# Autodesk Inventor assembly: Pakiet_zagrzany_same_ogniwa
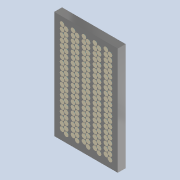
[picture p0: Inventor's stored thumbnail of the model, 180x180]
Saved by Autodesk Inventor 2021.3 (Build 253353000, 353)
## iProperties
Created: 2023-05-23
Part Number: Pakiet_zagrzany_same_ogniwa
Document SubType Name: Assembly
Designer: User
Author: User
## Documents named in this file (3)
- E:\Inventor\Projekty\Modele Robotyzacja Procesów\Pakiet_zagrzany_same_ogniwa.iam
- E:\Inventor\Projekty\Modele Robotyzacja Procesów\Model_Sita.ipt
- E:\Inventor\Projekty\Modele Robotyzacja Procesów\Model_Ogniwa.ipt
## Components (201 placed, 2 different names)
1. Model_Sita:1 — Zestawiające:1, Równoległe:1, Zestawiające:2, Równoległe:2
2. Model_Ogniwa:1 — Zestawiające:1, Równoległe:1
3. Model_Ogniwa:2
4. Model_Ogniwa:3
5. Model_Ogniwa:4
6. Model_Ogniwa:5
7. Model_Ogniwa:6
8. Model_Ogniwa:7
9. Model_Ogniwa:8
10. Model_Ogniwa:9
11. Model_Ogniwa:10
12. Model_Ogniwa:11
13. Model_Ogniwa:12
14. Model_Ogniwa:13
15. Model_Ogniwa:14
16. Model_Ogniwa:15
17. Model_Ogniwa:16
18. Model_Ogniwa:17
19. Model_Ogniwa:18
20. Model_Ogniwa:19
21. Model_Ogniwa:20
22. Model_Ogniwa:21
23. Model_Ogniwa:22
24. Model_Ogniwa:23
25. Model_Ogniwa:24
26. Model_Ogniwa:25
27. Model_Ogniwa:26
28. Model_Ogniwa:27
29. Model_Ogniwa:28
30. Model_Ogniwa:29
31. Model_Ogniwa:30
32. Model_Ogniwa:31
33. Model_Ogniwa:32
34. Model_Ogniwa:33
35. Model_Ogniwa:34
36. Model_Ogniwa:35
37. Model_Ogniwa:36
38. Model_Ogniwa:37
39. Model_Ogniwa:38
40. Model_Ogniwa:39
41. Model_Ogniwa:40
42. Model_Ogniwa:41
43. Model_Ogniwa:42
44. Model_Ogniwa:43
45. Model_Ogniwa:44
46. Model_Ogniwa:45
47. Model_Ogniwa:46
48. Model_Ogniwa:47
49. Model_Ogniwa:48
50. Model_Ogniwa:49
51. Model_Ogniwa:50
52. Model_Ogniwa:51
53. Model_Ogniwa:52
54. Model_Ogniwa:53
55. Model_Ogniwa:54
56. Model_Ogniwa:55
57. Model_Ogniwa:56
58. Model_Ogniwa:57
59. Model_Ogniwa:58
60. Model_Ogniwa:59
61. Model_Ogniwa:60
62. Model_Ogniwa:61
63. Model_Ogniwa:62
64. Model_Ogniwa:63
65. Model_Ogniwa:64
66. Model_Ogniwa:65
67. Model_Ogniwa:66
68. Model_Ogniwa:67
69. Model_Ogniwa:68
70. Model_Ogniwa:69
71. Model_Ogniwa:70
72. Model_Ogniwa:71
73. Model_Ogniwa:72
74. Model_Ogniwa:73
75. Model_Ogniwa:74
76. Model_Ogniwa:75
77. Model_Ogniwa:76
78. Model_Ogniwa:77
79. Model_Ogniwa:78
80. Model_Ogniwa:79
81. Model_Ogniwa:80
82. Model_Ogniwa:81
83. Model_Ogniwa:82
84. Model_Ogniwa:83
85. Model_Ogniwa:84
86. Model_Ogniwa:85
87. Model_Ogniwa:86
88. Model_Ogniwa:87
89. Model_Ogniwa:88
90. Model_Ogniwa:89
91. Model_Ogniwa:90
92. Model_Ogniwa:91
93. Model_Ogniwa:92
94. Model_Ogniwa:93
95. Model_Ogniwa:94
96. Model_Ogniwa:95
97. Model_Ogniwa:96
98. Model_Ogniwa:97
99. Model_Ogniwa:98
100. Model_Ogniwa:99
101. Model_Ogniwa:100
102. Model_Ogniwa:101 — Zestawiające:2, Równoległe:2
103. Model_Ogniwa:102
104. Model_Ogniwa:103
105. Model_Ogniwa:104
106. Model_Ogniwa:105
107. Model_Ogniwa:106
108. Model_Ogniwa:107
109. Model_Ogniwa:108
110. Model_Ogniwa:109
111. Model_Ogniwa:110
112. Model_Ogniwa:111
113. Model_Ogniwa:112
114. Model_Ogniwa:113
115. Model_Ogniwa:114
116. Model_Ogniwa:115
117. Model_Ogniwa:116
118. Model_Ogniwa:117
119. Model_Ogniwa:118
120. Model_Ogniwa:119
121. Model_Ogniwa:120
122. Model_Ogniwa:121
123. Model_Ogniwa:122
124. Model_Ogniwa:123
125. Model_Ogniwa:124
126. Model_Ogniwa:125
127. Model_Ogniwa:126
128. Model_Ogniwa:127
129. Model_Ogniwa:128
130. Model_Ogniwa:129
131. Model_Ogniwa:130
132. Model_Ogniwa:131
133. Model_Ogniwa:132
134. Model_Ogniwa:133
135. Model_Ogniwa:134
136. Model_Ogniwa:135
137. Model_Ogniwa:136
138. Model_Ogniwa:137
139. Model_Ogniwa:138
140. Model_Ogniwa:139
141. Model_Ogniwa:140
142. Model_Ogniwa:141
143. Model_Ogniwa:142
144. Model_Ogniwa:143
145. Model_Ogniwa:144
146. Model_Ogniwa:145
147. Model_Ogniwa:146
148. Model_Ogniwa:147
149. Model_Ogniwa:148
150. Model_Ogniwa:149
151. Model_Ogniwa:150
152. Model_Ogniwa:151
153. Model_Ogniwa:152
154. Model_Ogniwa:153
155. Model_Ogniwa:154
156. Model_Ogniwa:155
157. Model_Ogniwa:156
158. Model_Ogniwa:157
159. Model_Ogniwa:158
160. Model_Ogniwa:159
161. Model_Ogniwa:160
162. Model_Ogniwa:161
163. Model_Ogniwa:162
164. Model_Ogniwa:163
165. Model_Ogniwa:164
166. Model_Ogniwa:165
167. Model_Ogniwa:166
168. Model_Ogniwa:167
169. Model_Ogniwa:168
170. Model_Ogniwa:169
171. Model_Ogniwa:170
172. Model_Ogniwa:171
173. Model_Ogniwa:172
174. Model_Ogniwa:173
175. Model_Ogniwa:174
176. Model_Ogniwa:175
177. Model_Ogniwa:176
178. Model_Ogniwa:177
179. Model_Ogniwa:178
180. Model_Ogniwa:179
181. Model_Ogniwa:180
182. Model_Ogniwa:181
183. Model_Ogniwa:182
184. Model_Ogniwa:183
185. Model_Ogniwa:184
186. Model_Ogniwa:185
187. Model_Ogniwa:186
188. Model_Ogniwa:187
189. Model_Ogniwa:188
190. Model_Ogniwa:189
191. Model_Ogniwa:190
192. Model_Ogniwa:191
193. Model_Ogniwa:192
194. Model_Ogniwa:193
195. Model_Ogniwa:194
196. Model_Ogniwa:195
197. Model_Ogniwa:196
198. Model_Ogniwa:197
199. Model_Ogniwa:198
200. Model_Ogniwa:199
201. Model_Ogniwa:200
## Component patterns: (5 elements), (5 elements), (20 elements, first: Model_Ogniwa:1), Szyk komponentów 1:2 (20 elements), Szyk komponentów 1:3 (20 elements), Szyk komponentów 1:4 (20 elements), Szyk komponentów 1:5 (20 elements), (20 elements, first: Model_Ogniwa:101), Szyk komponentów 3:2 (20 elements), Szyk komponentów 3:3 (20 elements), Szyk komponentów 3:4 (20 elements), Szyk komponentów 3:5 (20 elements)
## Relationships (4: Mate 2, Flush 2)
- Zestawiające:1 [Mate]: Model_Sita:1 ↔ Model_Ogniwa:1
- Równoległe:1 [Flush]: Model_Sita:1 ↔ Model_Ogniwa:1
- Zestawiające:2 [Mate]: Model_Sita:1 ↔ Model_Ogniwa:101
- Równoległe:2 [Flush]: Model_Sita:1 ↔ Model_Ogniwa:101
